# Autodesk Inventor assembly: TPA
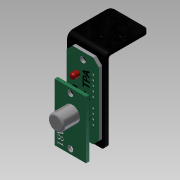
[picture p0: Inventor's stored thumbnail of the model, 180x180]
Saved by Autodesk Inventor 2015 SP1 (Build 190203100, 203)
## iProperties
Created: 2015-02-03
Part Number: TPA
Document SubType Name: Assembly
Designer: Rafi Kurnia Putra
Author: Rafi Kurnia Putra
## Documents named in this file (4)
- D:\Dropbox\krpai berkaki trui 2015\ROBUSTA\MEKANIK\ROBUSTA\Assembly TPA.iam
- D:\Dropbox\krpai berkaki trui 2015\ROBUSTA\MEKANIK\ROBUSTA\Dudukan TPA.ipt
- D:\Dropbox\krpai berkaki trui 2015\ROBUSTA\MEKANIK\ROBUSTA\Driver TPA.ipt
- D:\Dropbox\krpai berkaki trui 2015\ROBUSTA\MEKANIK\ROBUSTA\TPA81.ipt
## Components (3 placed, 3 different names)
1. Dudukan TPA:1 — Mate:7, Mate:8, Mate:9
2. Driver TPA:1 — Mate:4, Mate:5, Mate:6, Mate:7, Mate:8, Mate:9
3. TPA81:1 — Mate:4, Mate:5, Mate:6
## Relationships (6: Mate 6)
- Mate:4: Driver TPA:1 ↔ TPA81:1
- Mate:5: Driver TPA:1 ↔ TPA81:1
- Mate:6: Driver TPA:1 ↔ TPA81:1
- Mate:7: Dudukan TPA:1 ↔ Driver TPA:1
- Mate:8: Dudukan TPA:1 ↔ Driver TPA:1
- Mate:9: Dudukan TPA:1 ↔ Driver TPA:1
